# Autodesk Inventor assembly: GripperMount
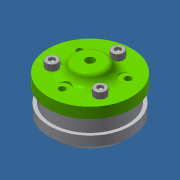
[picture p0: Inventor's stored thumbnail of the model, 180x180]
Saved by Autodesk Inventor 2016 (Build 200138000, 138)
## iProperties
Created: 2015-09-10
Part Number: GripperMount
Material: Generisch
Document SubType Name: Assembly
Designer: 4ndreas
Mass: 23.8121 g
Surface Area: 129.135 cm^2
Volume: 17.5511 cm^3
Density: 1.35673 g/cm^3
Author: 4ndreas
## Documents named in this file (6)
- C:\Users\4ndreas\Documents\Inventor\RobotARM v2\v4\_assemblys\GripperMount.iam
- C:\Users\4ndreas\Documents\Inventor\RobotARM v2\v4\_printed parts\GripperMountPlate.ipt
- C:\Users\4ndreas\Documents\Inventor\RobotARM v2\v4\_printed parts\GripperMount_b.ipt
- C:\Users\4ndreas\Documents\Inventor\RobotARM v2\v4\_printed parts\GripperMountPlatehock.ipt
- C:\Users\4ndreas\Documents\Inventor\RobotARM v2\v4\_standard Parts\Distanzhuelse_M3x5mm.ipt
- C:\Users\4ndreas\Documents\Inventor\Content Center Files\R2014\de-DE\DIN 912\DIN 912 - M3 x 0,5 x 16 x 14,75.ipt
## Components (9 placed, 5 different names)
1. GripperMount_b:1 — Fluchtend:1, Fluchtend:2, Fluchtend:3, Passend:1, Fluchtend:4, Passend:2, Passend:3, Passend:6, Passend:7, Passend:8, Passend:9, Passend:10, Passend:11, Passend:12, Passend:13, Passend:14, Passend:15, Passend:16, Passend:17
2. GripperMountPlate:1 — Fluchtend:4, Passend:2, Passend:3, Passend:4, Passend:5, Fluchtend:5, Passend:18, Passend:20
3. GripperMountPlatehock:1 — Passend:4, Passend:5, Fluchtend:5, Passend:19
4. Distanzhuelse_M3x5mm:1 — Passend:7, Passend:10, Passend:14
5. Distanzhuelse_M3x5mm:2 — Passend:8, Passend:11, Passend:13
6. Distanzhuelse_M3x5mm:3 — Passend:6, Passend:9, Passend:12
7. DIN 912 - ersetzt durch DIN EN ISO 4762 M3 x 16:1 — Passend:17, Passend:20
8. DIN 912 - ersetzt durch DIN EN ISO 4762 M3 x 16:2 — Passend:16, Passend:18
9. DIN 912 - ersetzt durch DIN EN ISO 4762 M3 x 16:3 — Passend:15, Passend:19
## Relationships (25: Mate 20, Flush 5)
- Fluchtend:1 [Flush]: GripperMount_b:1
- Fluchtend:2 [Flush]: GripperMount_b:1
- Fluchtend:3 [Flush]: GripperMount_b:1
- Passend:1 [Mate]: GripperMount_b:1
- Fluchtend:4 [Flush]: GripperMount_b:1 ↔ GripperMountPlate:1
- Passend:2 [Mate]: GripperMount_b:1 ↔ GripperMountPlate:1
- Passend:3 [Mate]: GripperMount_b:1 ↔ GripperMountPlate:1
- Passend:4 [Mate]: GripperMountPlate:1 ↔ GripperMountPlatehock:1
- Passend:5 [Mate]: GripperMountPlate:1 ↔ GripperMountPlatehock:1
- Fluchtend:5 [Flush]: GripperMountPlate:1 ↔ GripperMountPlatehock:1
- Passend:6 [Mate]: GripperMount_b:1 ↔ Distanzhuelse_M3x5mm:3
- Passend:7 [Mate]: GripperMount_b:1 ↔ Distanzhuelse_M3x5mm:1
- Passend:8 [Mate]: GripperMount_b:1 ↔ Distanzhuelse_M3x5mm:2
- Passend:9 [Mate]: GripperMount_b:1 ↔ Distanzhuelse_M3x5mm:3
- Passend:10 [Mate]: GripperMount_b:1 ↔ Distanzhuelse_M3x5mm:1
- Passend:11 [Mate]: GripperMount_b:1 ↔ Distanzhuelse_M3x5mm:2
- Passend:12 [Mate]: GripperMount_b:1 ↔ Distanzhuelse_M3x5mm:3
- Passend:13 [Mate]: GripperMount_b:1 ↔ Distanzhuelse_M3x5mm:2
- Passend:14 [Mate]: GripperMount_b:1 ↔ Distanzhuelse_M3x5mm:1
- Passend:15 [Mate]: GripperMount_b:1 ↔ DIN 912 - ersetzt durch DIN EN ISO 4762 M3 x 16:3
- Passend:16 [Mate]: GripperMount_b:1 ↔ DIN 912 - ersetzt durch DIN EN ISO 4762 M3 x 16:2
- Passend:17 [Mate]: GripperMount_b:1 ↔ DIN 912 - ersetzt durch DIN EN ISO 4762 M3 x 16:1
- Passend:18 [Mate]: GripperMountPlate:1 ↔ DIN 912 - ersetzt durch DIN EN ISO 4762 M3 x 16:2
- Passend:19 [Mate]: GripperMountPlatehock:1 ↔ DIN 912 - ersetzt durch DIN EN ISO 4762 M3 x 16:3
- Passend:20 [Mate]: GripperMountPlate:1 ↔ DIN 912 - ersetzt durch DIN EN ISO 4762 M3 x 16:1
